# Autodesk Inventor assembly: Tamale Assembly Plate V5 on Chuck
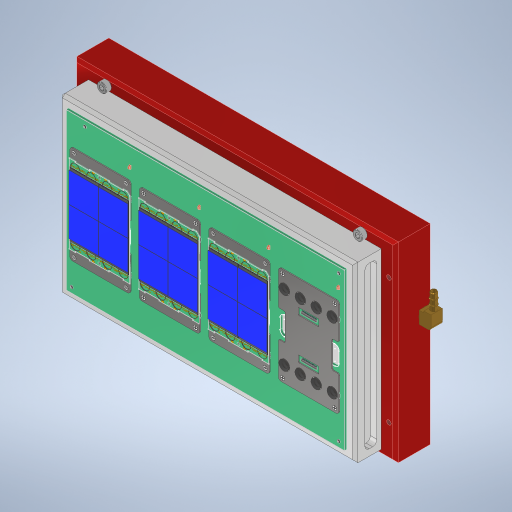
[picture p0: Inventor's stored thumbnail of the model, 512x512]
Saved by Autodesk Inventor 2023 (Build 270158000, 158)
## iProperties
Created: 2023-04-13
Part Number: Tamale Assembly Plate V5 on Chuck
Document SubType Name: Assembly
Designer: Caleb
Author: Caleb
## Documents named in this file (3)
- C:\Users\Caleb\Desktop\nebraska-silicon-lab\Hardware\ETL\Module Assembly\Tamale Assembly Plate V5\Tamale Assembly Plate V5 on Chuck.iam
- C:\Users\Caleb\Desktop\nebraska-silicon-lab\Hardware\ETL\Module Assembly\Chuck - V2\Chuck - V2.iam
- C:\Users\Caleb\Desktop\nebraska-silicon-lab\Hardware\ETL\Module Assembly\Tamale Assembly Plate V5\Tamale Assembly Plate Assembly V5.iam
## Components (2 placed, 2 different names)
1. Chuck - V2:1 [sub-assembly] — Mate:1, Tangent:1, Tangent:2, Tangent:3
2. Tamale Assembly Plate Assembly V5:1 [sub-assembly] — Mate:1, Tangent:1, Tangent:2, Tangent:3
## Relationships (4: Tangent 3, Mate 1)
- Mate:1: Chuck - V2:1 ↔ Tamale Assembly Plate Assembly V5:1
- Tangent:1: Chuck - V2:1 ↔ Tamale Assembly Plate Assembly V5:1
- Tangent:2: Chuck - V2:1 ↔ Tamale Assembly Plate Assembly V5:1
- Tangent:3: Chuck - V2:1 ↔ Tamale Assembly Plate Assembly V5:1
